# Autodesk Inventor assembly: Complete Roller Pneumatic Cylinder Assembly
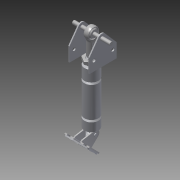
[picture p0: Inventor's stored thumbnail of the model, 180x180]
Saved by Autodesk Inventor 2014 (Build 180170000, 170)
## iProperties
Created: 2014-01-18
Part Number: Complete Roller Pneumatic Cylinder Assembly
Document SubType Name: Assembly
Designer: Michael
Author: Michael
## Documents named in this file (7)
- C:\Users\Michael\Documents\GitHub\2014buildCAD\New Collector\Complete Roller Pneumatic Cylinder Assembly.iam
- C:\Users\Michael\Documents\GitHub\2014buildCAD\New Collector\6498K602 Pneumatic Cylinder Assembly.iam
- C:\Users\Michael\Documents\GitHub\2014buildCAD\New Collector\Axle 0.190 in 3 in length.ipt
- C:\Users\Michael\Documents\GitHub\2014buildCAD\New Collector\Bracket.ipt
- C:\Users\Michael\Documents\GitHub\2014buildCAD\New Collector\Rod End (McMaster Part #6498K592).ipt
- C:\Users\Michael\Documents\GitHub\2014buildCAD\New Collector\Roller Pneumatic Back Connector (Custom).ipt
- C:\Users\Michael\Documents\GitHub\2014buildCAD\New Collector\Foot Bracket Mount (McMaster Part #6498K710).ipt
## Components (7 placed, 6 different names)
1. 6498K602 Pneumatic Cylinder Assembly:1 [sub-assembly] — Mate:1, Mate:2, Mate:3, Mate:4
2. Axle 0.190 in 3 in length:1 — Mate:5, Mate:6, Mate:7, Flush:1
3. Bracket:1 — Mate:6, Mate:8, Mate:9, Mate:10, Flush:1, Angle:1
4. Rod End (McMaster Part #6498K592):1 — Mate:1, Mate:2, Mate:5, Mate:9
5. Roller Pneumatic Back Connector (Custom):1 — Mate:11, Mate:12, Mate:13
6. Foot Bracket Mount (McMaster Part #6498K710):1 — Mate:3, Mate:4, Mate:11, Mate:12, Mate:13, Angle:1
7. Bracket:2 — Mate:7, Mate:8, Mate:10
## Relationships (15: Mate 13, Flush 1, Angle 1)
- Mate:1: 6498K602 Pneumatic Cylinder Assembly:1 ↔ Rod End (McMaster Part #6498K592):1
- Mate:2: 6498K602 Pneumatic Cylinder Assembly:1 ↔ Rod End (McMaster Part #6498K592):1
- Mate:3: 6498K602 Pneumatic Cylinder Assembly:1 ↔ Foot Bracket Mount (McMaster Part #6498K710):1
- Mate:4: 6498K602 Pneumatic Cylinder Assembly:1 ↔ Foot Bracket Mount (McMaster Part #6498K710):1
- Mate:5: Axle 0.190 in 3 in length:1 ↔ Rod End (McMaster Part #6498K592):1
- Mate:6: Axle 0.190 in 3 in length:1 ↔ Bracket:1
- Mate:7: Axle 0.190 in 3 in length:1 ↔ Bracket:2
- Mate:8 (25.4 mm): Bracket:1 ↔ Bracket:2
- Mate:9 (8.7376 mm): Bracket:1 ↔ Rod End (McMaster Part #6498K592):1
- Mate:10: Bracket:1 ↔ Bracket:2
- Mate:11: Roller Pneumatic Back Connector (Custom):1 ↔ Foot Bracket Mount (McMaster Part #6498K710):1
- Mate:12: Roller Pneumatic Back Connector (Custom):1 ↔ Foot Bracket Mount (McMaster Part #6498K710):1
- Flush:1 (-9.525 mm): Axle 0.190 in 3 in length:1 ↔ Bracket:1
- Mate:13: Roller Pneumatic Back Connector (Custom):1 ↔ Foot Bracket Mount (McMaster Part #6498K710):1
- Angle:1 (90 deg): Bracket:1 ↔ Foot Bracket Mount (McMaster Part #6498K710):1
